# Autodesk Inventor assembly: fan_heatsink
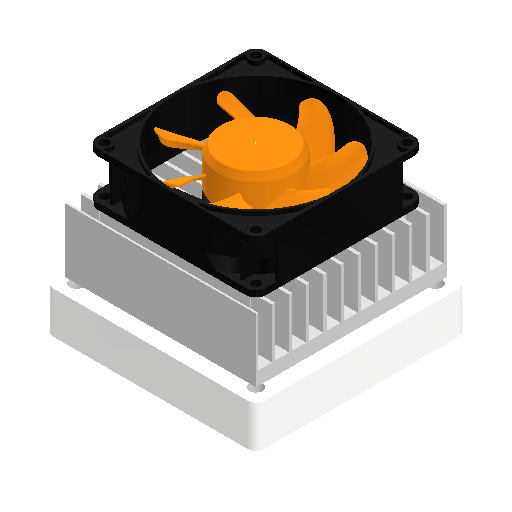
[picture p0: Inventor's stored thumbnail of the model, 512x512]
Saved by Autodesk Inventor 2026.2 (Build 302298010, 298A)
## iProperties
Created: 2026-04-29
Part Number: fan_heatsink
Document SubType Name: Assembly
Designer: danie
Author: danie
## Documents named in this file (6)
- C:\Users\danie\OneDrive\Documentos\Inventor\Arbol\V4\V4\thermalmodule\fan_heatsink.iam
- C:\Users\danie\OneDrive\Documentos\Inventor\Arbol\V4\V4\thermalmodule\peltier.ipt
- C:\Users\danie\OneDrive\Documentos\Inventor\Arbol\V4\V4\aluminum-heatsink\heatsink\heatsink\heatsink.ipt
- C:\Users\danie\OneDrive\Documentos\Inventor\Arbol\V4\V4\dc-fan-80-x-80-x-25-mm-1.snapshot.1\DC FAN 80 X 80 X 25\DC FAN 80 X 80 X 25\DC FAN 80 X 80 X 25.iam
- C:\Users\danie\OneDrive\Documentos\Inventor\Arbol\V4\V4\thermalmodule\inf_soporte.ipt
- C:\Users\danie\OneDrive\Documentos\Inventor\Arbol\V4\V4\thermalmodule\sup_soporte.ipt
## Components (5 placed, 5 different names)
1. peltier:1 — Mate:2, Mate:8, Mate:9, Mate:10, Mate:11, Mate:12, Mate:14
2. heatsink:1 — Mate:1, Mate:4, Mate:5, Mate:7, Mate:14
3. DC FAN 80 X 80 X 25:1 [sub-assembly] — Mate:1, Mate:3, Mate:4, Mate:5, Mate:7, Mate:8
4. inf_soporte:1 — Mate:9, Mate:10, Mate:12, Mate:13, Flush:1, Flush:2
5. sup_soporte:1 — Mate:13, Flush:1, Flush:2
## Relationships (15: Mate 13, Flush 2)
- Mate:1: heatsink:1 ↔ DC FAN 80 X 80 X 25:1
- Mate:2: peltier:1
- Mate:3: DC FAN 80 X 80 X 25:1
- Mate:4: heatsink:1 ↔ DC FAN 80 X 80 X 25:1
- Mate:5: heatsink:1 ↔ DC FAN 80 X 80 X 25:1
- Mate:7: heatsink:1 ↔ DC FAN 80 X 80 X 25:1
- Mate:8: peltier:1 ↔ DC FAN 80 X 80 X 25:1
- Mate:9: peltier:1 ↔ inf_soporte:1
- Mate:10: peltier:1 ↔ inf_soporte:1
- Mate:11: peltier:1
- Mate:12: peltier:1 ↔ inf_soporte:1
- Mate:13: inf_soporte:1 ↔ sup_soporte:1
- Flush:1: inf_soporte:1 ↔ sup_soporte:1
- Flush:2: inf_soporte:1 ↔ sup_soporte:1
- Mate:14: peltier:1 ↔ heatsink:1
